# Autodesk Inventor assembly: Body_assemb
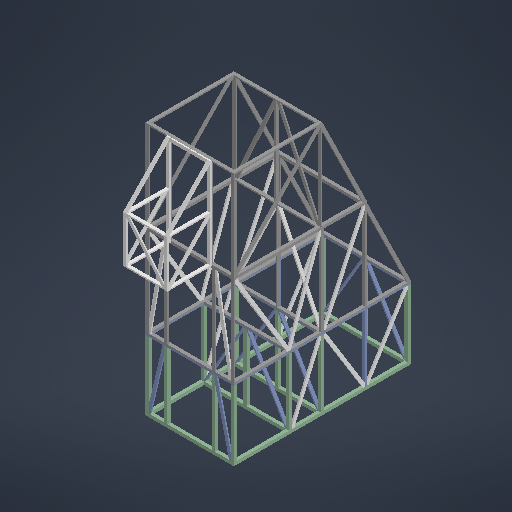
[picture p0: Inventor's stored thumbnail of the model, 512x512]
Saved by Autodesk Inventor 2026 (Build 300175000, 175)
## iProperties
Created: 2025-08-28
Part Number: Body_assemb
Document SubType Name: Assembly
Designer: trott
Author: trott
## Documents named in this file (4)
- C:\Users\trott\Documents\UofSC-ASME-Tiger-Burn-Design-2025\CAD\Assembly\Base_assemb.iam
- C:\Users\trott\Documents\UofSC-ASME-Tiger-Burn-Design-2025\CAD\Body\Base 01\Base 01.iam
- C:\Users\trott\Documents\UofSC-ASME-Tiger-Burn-Design-2025\CAD\Body\Base 02\Base 02.iam
- C:\Users\trott\Documents\UofSC-ASME-Tiger-Burn-Design-2025\CAD\Body\Base 03\Base 03.iam
## Components (3 placed, 3 different names)
1. Base 01:1 [sub-assembly] — Mate:1, Flush:1, Flush:2
2. Base 02:1 [sub-assembly] — Mate:1, Flush:1, Flush:2, Mate:2, Flush:3, Flush:4
3. Base 03:1 [sub-assembly] — Mate:2, Flush:3, Flush:4
## Relationships (6: Flush 4, Mate 2)
- Mate:1: Base 01:1 ↔ Base 02:1
- Flush:1: Base 01:1 ↔ Base 02:1
- Flush:2: Base 01:1 ↔ Base 02:1
- Mate:2: Base 02:1 ↔ Base 03:1
- Flush:3: Base 02:1 ↔ Base 03:1
- Flush:4: Base 02:1 ↔ Base 03:1
